# Autodesk Inventor assembly: Par_Man
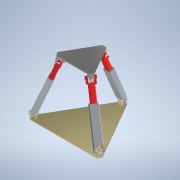
[picture p0: Inventor's stored thumbnail of the model, 180x180]
Saved by Autodesk Inventor 2021 (Build 250183000, 183)
## iProperties
Created: 2020-12-13
Part Number: Par_Man
Document SubType Name: Assembly
Designer: Ashiqrahman
Author: Ashiqrahman
Source: UnKnown
## Documents named in this file (6)
- D:\projects\borewell\parallel manipulator grabcad\Imported Components\Ass\Ass.iam
- D:\projects\borewell\parallel manipulator grabcad\Imported Components\Ass\base_CATPart.ipt
- D:\projects\borewell\parallel manipulator grabcad\Imported Components\Ass\cardan.ipt
- D:\projects\borewell\parallel manipulator grabcad\Imported Components\Ass\actor_base_CATPart.ipt
- D:\projects\borewell\parallel manipulator grabcad\Imported Components\Ass\extension_CATPart.ipt
- D:\projects\borewell\parallel manipulator grabcad\Imported Components\Ass\upper_base_CAT.ipt
## Components (14 placed, 14 different names)
1. base_AllCATPart.2 — Mate:7, Mate:8, Mate:18, Mate:19, Mate:29, Mate:31
2. Cardan_AllCATPart.3 — Mate:20, Mate:21, Mate:22, Mate:23
3. Cardan_AllCATPart.4 — Mate:7, Mate:8, Mate:9, Mate:30
4. Cardan_AllCATPart.5 — Mate:1, Mate:2, Mate:3, Mate:4
5. Cardan_AllCATPart.6 — Mate:16, Mate:17, Mate:18, Mate:19
6. Cardan_AllCATPart.7 — Mate:10, Mate:11, Mate:12, Mate:13
7. Cardan_AllCATPart.2 — Mate:26, Mate:27, Mate:29, Mate:31
8. actor_base_AllCATPart.4 — Mate:5, Mate:6, Mate:9, Mate:30
9. actor_base_AllCATPart.1 — Mate:24, Mate:25, Mate:26, Mate:27
10. actor_base_AllCATPart.3 — Mate:14, Mate:15, Mate:16, Mate:17
11. Extension_AllCATPart.3 — Mate:1, Mate:2, Mate:5, Mate:6
12. Extension_AllCATPart.1 — Mate:20, Mate:21, Mate:24, Mate:25
13. Extension_AllCATPart.2 — Mate:10, Mate:11, Mate:14, Mate:15
14. upper_base_CATPart.1 — Mate:3, Mate:4, Mate:12, Mate:13, Mate:22, Mate:23
## Relationships (30: Mate 30)
- Mate:1: Cardan_AllCATPart.5 ↔ Extension_AllCATPart.3
- Mate:2: Cardan_AllCATPart.5 ↔ Extension_AllCATPart.3
- Mate:3: Cardan_AllCATPart.5 ↔ upper_base_CATPart.1
- Mate:4: Cardan_AllCATPart.5 ↔ upper_base_CATPart.1
- Mate:5: actor_base_AllCATPart.4 ↔ Extension_AllCATPart.3
- Mate:6: actor_base_AllCATPart.4 ↔ Extension_AllCATPart.3
- Mate:7: base_AllCATPart.2 ↔ Cardan_AllCATPart.4
- Mate:8: base_AllCATPart.2 ↔ Cardan_AllCATPart.4
- Mate:9: Cardan_AllCATPart.4 ↔ actor_base_AllCATPart.4
- Mate:10: Cardan_AllCATPart.7 ↔ Extension_AllCATPart.2
- Mate:11: Cardan_AllCATPart.7 ↔ Extension_AllCATPart.2
- Mate:12: Cardan_AllCATPart.7 ↔ upper_base_CATPart.1
- Mate:13: Cardan_AllCATPart.7 ↔ upper_base_CATPart.1
- Mate:14: actor_base_AllCATPart.3 ↔ Extension_AllCATPart.2
- Mate:15: actor_base_AllCATPart.3 ↔ Extension_AllCATPart.2
- Mate:16: Cardan_AllCATPart.6 ↔ actor_base_AllCATPart.3
- Mate:17: Cardan_AllCATPart.6 ↔ actor_base_AllCATPart.3
- Mate:18: base_AllCATPart.2 ↔ Cardan_AllCATPart.6
- Mate:19: base_AllCATPart.2 ↔ Cardan_AllCATPart.6
- Mate:20: Cardan_AllCATPart.3 ↔ Extension_AllCATPart.1
- Mate:21: Cardan_AllCATPart.3 ↔ Extension_AllCATPart.1
- Mate:22: Cardan_AllCATPart.3 ↔ upper_base_CATPart.1
- Mate:23: Cardan_AllCATPart.3 ↔ upper_base_CATPart.1
- Mate:24: actor_base_AllCATPart.1 ↔ Extension_AllCATPart.1
- Mate:25: actor_base_AllCATPart.1 ↔ Extension_AllCATPart.1
- Mate:26: Cardan_AllCATPart.2 ↔ actor_base_AllCATPart.1
- Mate:27: Cardan_AllCATPart.2 ↔ actor_base_AllCATPart.1
- Mate:29: base_AllCATPart.2 ↔ Cardan_AllCATPart.2
- Mate:30: Cardan_AllCATPart.4 ↔ actor_base_AllCATPart.4
- Mate:31: base_AllCATPart.2 ↔ Cardan_AllCATPart.2
